# Autodesk Inventor assembly: Pallet Assembly
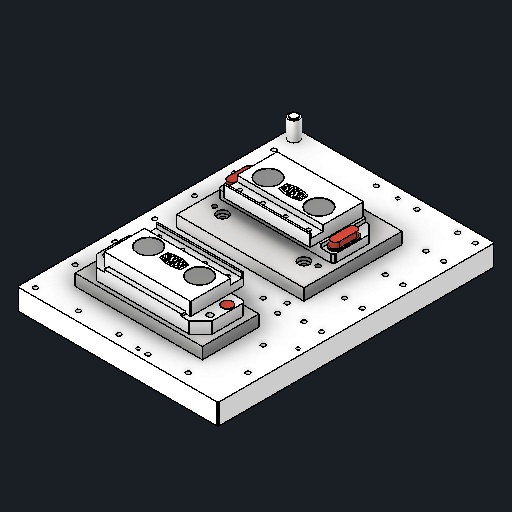
[picture p0: Inventor's stored thumbnail of the model, 512x512]
Saved by Autodesk Inventor 2026.2 (Build 302298000, 298)
## iProperties
Created: 2026-04-18
Part Number: Pallet Assembly
Document SubType Name: Assembly
Designer: JoshuaEah
Author: JoshuaEah
## Documents named in this file (6)
- C:\Users\JoshuaEah\Documents\GitHub\Designed-Trinkets\Makera Carvera Air Pallet\Pallet Assembly.iam
- C:\Users\JoshuaEah\Documents\GitHub\Designed-Trinkets\Makera Carvera Air Pallet\Table.ipt
- C:\Users\JoshuaEah\Documents\GitHub\Designed-Trinkets\Makera Carvera Air Pallet\Mod Vises\Fixed Side Assembly.iam
- C:\Users\JoshuaEah\Documents\GitHub\Designed-Trinkets\Makera Carvera Air Pallet\Mod Vises\Adjustable Side Assembly.iam
- C:\Users\JoshuaEah\Documents\GitHub\Designed-Trinkets\Makera Carvera Air Pallet\Fixed Side Adapter Plate.ipt
- C:\Users\JoshuaEah\Documents\GitHub\Designed-Trinkets\Makera Carvera Air Pallet\Adjustable Side Adapter Plate.ipt
## Components (5 placed, 5 different names)
1. Table:1 — Insert:1, Insert:2, Adj. Side Base Pos 1, Adj. Side Base Pos 2
2. Fixed Side Assembly:1 [sub-assembly] — Mate:1, Mate:2
3. Adjustable Side Assembly:1 [sub-assembly] — Adj. Side Pos 1, Adj. Side Pos 2, Adj. Side Pos 3
4. Fixed Side Adapter Plate:1 — Insert:1, Insert:2, Mate:1, Mate:2
5. Adjustable Side Adapter Plate:1 — Adj. Side Pos 1, Adj. Side Pos 2, Adj. Side Pos 3, Adj. Side Base Pos 1, Adj. Side Base Pos 2
## Relationships (9: Insert 4, TranslationJoint 3, Mate 2)
- Insert:1: Table:1 ↔ Fixed Side Adapter Plate:1
- Insert:2: Table:1 ↔ Fixed Side Adapter Plate:1
- Mate:1: Fixed Side Assembly:1 ↔ Fixed Side Adapter Plate:1
- Mate:2: Fixed Side Assembly:1 ↔ Fixed Side Adapter Plate:1
- Adj. Side Pos 1 [TranslationJoint]: Adjustable Side Assembly:1 ↔ Adjustable Side Adapter Plate:1
- Adj. Side Pos 2 [TranslationJoint]: Adjustable Side Assembly:1 ↔ Adjustable Side Adapter Plate:1
- Adj. Side Pos 3 [TranslationJoint]: Adjustable Side Assembly:1 ↔ Adjustable Side Adapter Plate:1
- Adj. Side Base Pos 1 [Insert]: Table:1 ↔ Adjustable Side Adapter Plate:1
- Adj. Side Base Pos 2 [Insert]: Table:1 ↔ Adjustable Side Adapter Plate:1
## Named parameters: openingWidth = 76.2 mm
